# Autodesk Inventor assembly: ASSY,INTAKE
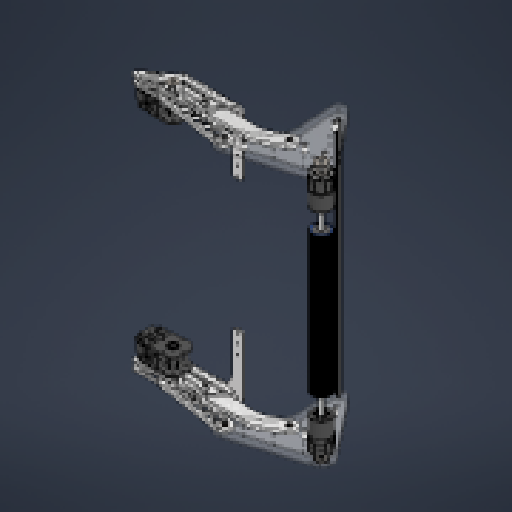
[picture p0: Inventor's stored thumbnail of the model, 512x512]
Saved by Autodesk Inventor 2026.1 (Build 301233020, 233B)
## iProperties
Created: 2026-02-09
Part Number: ASSY,INTAKE
Document SubType Name: Assembly
Designer: Jthib
Mass: 4084.96 g
Surface Area: 8083.76 cm^2
Volume: 1639.15 cm^3
Density: 2.49213 g/cm^3
Author: Jthib
## Documents named in this file (19)
- C:\Users\Owen\Documents\GitHub\2026-Robot-Mechanical\Intake\ASSY,INTAKE.iam
- C:\Users\Owen\Documents\GitHub\2026-Robot-Mechanical\Intake\PLATE,INTAKE,SIDE.ipt
- C:\Users\Owen\Documents\GitHub\2026-Robot-Mechanical\#1_CAD Library\Power Transmission\Bearings\PURCHASED,HEX_BEARING.ipt
- C:\Users\Owen\Documents\GitHub\2026-Robot-Mechanical\Intake\3DPRINT,INTAKE,SPACER.ipt
- C:\Users\Owen\Documents\GitHub\2026-Robot-Mechanical\Intake\STOCK,HEX,INTAKE.ipt
- C:\Users\Owen\Documents\GitHub\2026-Robot-Mechanical\Intake\PURCHASED,92320A546_18-8 Stainless Steel Unthreaded Spacer.ipt
- C:\Users\Owen\Documents\GitHub\2026-Robot-Mechanical\#1_CAD Library\Electronics\CONTROLS,SPARK_FLEX.ipt
- C:\Users\Owen\Documents\GitHub\2026-Robot-Mechanical\#1_CAD Library\Motors\MOTOR,REV,NEO,VORTEX.ipt
- C:\Users\Owen\Documents\GitHub\2026-Robot-Mechanical\Intake\STOCK,CHURRO,LOWER,INTAKE.ipt
- C:\Users\Owen\Documents\GitHub\2026-Robot-Mechanical\Intake\PLATE,HINGE,INTAKE,FRONT.ipt
- C:\Users\Owen\Documents\GitHub\2026-Robot-Mechanical\Intake\PLATE,LINK,FRONT,INTAKE.ipt
- C:\Users\Owen\Documents\GitHub\2026-Robot-Mechanical\Intake\PLATE,LINK,REAR,INTAKE.ipt
- C:\Users\Owen\Documents\GitHub\2026-Robot-Mechanical\Intake\PURCHASED,20-1,90deg,MAX-PLANETARY.ipt
- C:\Users\Owen\Documents\GitHub\2026-Robot-Mechanical\Intake\PURCHASED,6391K186_Oil-Embedded 841 Bronze Sleeve Bearing.ipt
- C:\Users\Owen\Documents\GitHub\2026-Robot-Mechanical\Intake\PURCHASED,92390A271_18-8 Stainless Steel Clevis Pin.ipt
- C:\Users\Owen\Documents\GitHub\2026-Robot-Mechanical\Intake\3DPRINT,SPACER,HEX,INTAKE.ipt
- C:\Users\Owen\Documents\GitHub\2026-Robot-Mechanical\Intake\PURCHASED,2796T12_Ultra-Low-Friction Dry-Running Thrust Bearing.ipt
- C:\Users\Owen\Documents\GitHub\2026-Robot-Mechanical\Intake\PLATE,CLAMP,MK4i,Swerve,CUSTOM,FRC2026.ipt
- C:\Users\Owen\Documents\GitHub\2026-Robot-Mechanical\Intake\CAST,2inOD,ROLLER.ipt
## Components (56 placed, 18 different names)
1. PLATE,INTAKE,SIDE:1 — Symmetry:1, Insert:28, Insert:29, Insert:30, Mate:31
2. PLATE,INTAKE,SIDE:2 — Angle:3, Insert:27, Mate:30
3. 3DPRINT,INTAKE,SPACER:2 — Mate:31
4. 3DPRINT,INTAKE,SPACER:4
5. 3DPRINT,INTAKE,SPACER:5
6. 3DPRINT,INTAKE,SPACER:1
7. PLATE,INTAKE,SIDE:3 — Angle:2, Insert:26, Mate:27, Mate:28, Mate:29
8. PLATE,INTAKE,SIDE:4 — Symmetry:1, Mate:8, Mate:9, Mate:10, Insert:25, Mate:33, Mate:35, Mate:50
9. 3DPRINT,INTAKE,SPACER:7 — Mate:27, Mate:28
10. 3DPRINT,INTAKE,SPACER:10
11. 3DPRINT,INTAKE,SPACER:11
12. STOCK,HEX,INTAKE:1 — Flush:1, Mate:21, Mate:22, Mate:26, Mate:63, Mate:64, Mate:65
13. PURCHASED,92320A546_18-8 Stainless Steel Unthreaded Spacer:1 — Mate:8, Mate:43
14. PURCHASED,92320A546_18-8 Stainless Steel Unthreaded Spacer:2 — Mate:9, Mate:10, Mate:23, Mate:29, Mate:46
15. MOTOR,REV,NEO,VORTEX:1 — Angle:2
16. CONTROLS,SPARK_FLEX:1
17. MOTOR,REV,NEO,VORTEX:2
18. CONTROLS,SPARK_FLEX:2 — Angle:3, Mate:26
19. PURCHASED,HEX_BEARING:7 — Insert:25, Mate:21
20. PURCHASED,HEX_BEARING:8 — Insert:26
21. PURCHASED,HEX_BEARING:9 — Insert:27
22. PURCHASED,HEX_BEARING:10 — Insert:28, Mate:22
23. PURCHASED,92320A546_18-8 Stainless Steel Unthreaded Spacer:3 — Insert:30, Mate:61
24. PURCHASED,92320A546_18-8 Stainless Steel Unthreaded Spacer:4 — Insert:29, Mate:23, Mate:30, Mate:60
25. STOCK,CHURRO,LOWER,INTAKE:1
26. PLATE,HINGE,INTAKE,FRONT:1 — Mate:38, Mate:39, Mate:48, Mate:49, Insert:40, Mate:69, Mate:70, Mate:73
27. PLATE,LINK,FRONT,INTAKE:1 — Insert:33, Insert:36
28. PLATE,LINK,REAR,INTAKE:1 — Insert:34, Mate:41
29. PURCHASED,20-1,90deg,MAX-PLANETARY:1 — Mate:69, Mate:70, Mate:73
30. PURCHASED,6391K186_Oil-Embedded 841 Bronze Sleeve Bearing:1 — Insert:33, Mate:33, Mate:43
31. PURCHASED,92390A271_18-8 Stainless Steel Clevis Pin:1 — Insert:49, Mate:66
32. PLATE,HINGE,INTAKE,FRONT:2 — Mate:38, Mate:40, Insert:39, Mate:41, Mate:42, Mate:45, Mate:47, Insert:49
33. PURCHASED,6391K186_Oil-Embedded 841 Bronze Sleeve Bearing:2 — Insert:34, Mate:35, Mate:46
34. PURCHASED,HEX_BEARING:11 — Insert:39
35. PURCHASED,6391K186_Oil-Embedded 841 Bronze Sleeve Bearing:3 — Insert:36, Insert:37, Insert:38, Mate:66
36. 3DPRINT,SPACER,HEX,INTAKE:1 — Insert:40
37. PURCHASED,2796T12_Ultra-Low-Friction Dry-Running Thrust Bearing:1 — Insert:38, Mate:39
38. PURCHASED,2796T12_Ultra-Low-Friction Dry-Running Thrust Bearing:2 — Insert:37, Mate:40
39. PLATE,CLAMP,MK4i,Swerve,CUSTOM,FRC2026:1 — Mate:47, Mate:48, Mate:49, Mate:50, Flush:5, Mate:62
40. PLATE,CLAMP,MK4i,Swerve,CUSTOM,FRC2026:2 — Flush:5, Mate:57, Mate:58, Flush:7, Mate:62
41. PLATE,HINGE,INTAKE,FRONT:3 — Mate:51, Mate:52, Insert:41, Mate:57, Mate:58, Mate:71, Insert:51, Mate:72, Mate:74
42. PLATE,HINGE,INTAKE,FRONT:4 — Mate:51, Mate:52, Insert:42, Insert:43, Mate:56, Flush:7, Insert:50
43. PLATE,LINK,REAR,INTAKE:2 — Insert:46, Mate:56, Flush:4
44. PLATE,LINK,FRONT,INTAKE:2 — Insert:44, Insert:45, Flush:4
45. PURCHASED,6391K186_Oil-Embedded 841 Bronze Sleeve Bearing:4 — Insert:44, Mate:53, Mate:54, Mate:55
46. PURCHASED,6391K186_Oil-Embedded 841 Bronze Sleeve Bearing:5 — Insert:45, Mate:61
47. PURCHASED,6391K186_Oil-Embedded 841 Bronze Sleeve Bearing:6 — Insert:46, Mate:60
48. PURCHASED,2796T12_Ultra-Low-Friction Dry-Running Thrust Bearing:3 — Insert:41, Mate:54
49. PURCHASED,2796T12_Ultra-Low-Friction Dry-Running Thrust Bearing:4 — Insert:42, Mate:55
50. PURCHASED,92390A271_18-8 Stainless Steel Clevis Pin:2 — Insert:43, Mate:53
51. CAST,2inOD,ROLLER:1 — Mate:63, Mate:68
52. CAST,2inOD,ROLLER:2 — Mate:64, Mate:67, Mate:68
53. CAST,2inOD,ROLLER:3 — Mate:65, Mate:67
54. PURCHASED,20-1,90deg,MAX-PLANETARY:2 — Mate:71, Mate:72, Mate:74
55. PURCHASED,HEX_BEARING:12 — Insert:50
56. 3DPRINT,SPACER,HEX,INTAKE:2 — Insert:51
## Relationships (97: Mate 59, Insert 31, Flush 4, Angle 2, Symmetry 1)
- [Insert]: PLATE,INTAKE,SIDE:2 ↔ 3DPRINT,INTAKE,SPACER:1
- [Insert]: PLATE,INTAKE,SIDE:2 ↔ 3DPRINT,INTAKE,SPACER:2
- [Insert]: PLATE,INTAKE,SIDE:2 ↔ 3DPRINT,INTAKE,SPACER:4
- [Insert]: PLATE,INTAKE,SIDE:2 ↔ 3DPRINT,INTAKE,SPACER:5
- [Insert]: PLATE,INTAKE,SIDE:4 ↔ 3DPRINT,INTAKE,SPACER:7
- [Insert]: PLATE,INTAKE,SIDE:4 ↔ 3DPRINT,INTAKE,SPACER:10
- [Insert]: PLATE,INTAKE,SIDE:4 ↔ 3DPRINT,INTAKE,SPACER:11
- Symmetry:1: PLATE,INTAKE,SIDE:1 ↔ PLATE,INTAKE,SIDE:4
- Flush:1: STOCK,HEX,INTAKE:1
- [Mate]: PLATE,INTAKE,SIDE:3 ↔ PURCHASED,92320A546_18-8 Stainless Steel Unthreaded Spacer:1
- Mate:8: PLATE,INTAKE,SIDE:4 ↔ PURCHASED,92320A546_18-8 Stainless Steel Unthreaded Spacer:1
- Mate:9: PLATE,INTAKE,SIDE:4 ↔ PURCHASED,92320A546_18-8 Stainless Steel Unthreaded Spacer:2
- Mate:10: PLATE,INTAKE,SIDE:4 ↔ PURCHASED,92320A546_18-8 Stainless Steel Unthreaded Spacer:2
- [Mate]: MOTOR,REV,NEO,VORTEX:1 ↔ CONTROLS,SPARK_FLEX:1
- [Mate]: MOTOR,REV,NEO,VORTEX:1 ↔ CONTROLS,SPARK_FLEX:1
- [Mate]: MOTOR,REV,NEO,VORTEX:1 ↔ CONTROLS,SPARK_FLEX:1
- [Mate]: STOCK,HEX,INTAKE:1 ↔ CONTROLS,SPARK_FLEX:1
- [Mate]: PLATE,INTAKE,SIDE:3 ↔ CONTROLS,SPARK_FLEX:1
- [Mate]: MOTOR,REV,NEO,VORTEX:2 ↔ CONTROLS,SPARK_FLEX:2
- [Mate]: MOTOR,REV,NEO,VORTEX:2 ↔ CONTROLS,SPARK_FLEX:2
- [Mate]: MOTOR,REV,NEO,VORTEX:2 ↔ CONTROLS,SPARK_FLEX:2
- [Mate]: PLATE,INTAKE,SIDE:2 ↔ CONTROLS,SPARK_FLEX:2
- Angle:2 (0 deg): PLATE,INTAKE,SIDE:3 ↔ MOTOR,REV,NEO,VORTEX:1
- Angle:3 (0 deg): PLATE,INTAKE,SIDE:2 ↔ CONTROLS,SPARK_FLEX:2
- Insert:25: PLATE,INTAKE,SIDE:4 ↔ PURCHASED,HEX_BEARING:7
- Insert:26: PLATE,INTAKE,SIDE:3 ↔ PURCHASED,HEX_BEARING:8
- Insert:27: PLATE,INTAKE,SIDE:2 ↔ PURCHASED,HEX_BEARING:9
- Insert:28: PLATE,INTAKE,SIDE:1 ↔ PURCHASED,HEX_BEARING:10
- Mate:21: STOCK,HEX,INTAKE:1 ↔ PURCHASED,HEX_BEARING:7
- Mate:22: STOCK,HEX,INTAKE:1 ↔ PURCHASED,HEX_BEARING:10
- Insert:29: PLATE,INTAKE,SIDE:1 ↔ PURCHASED,92320A546_18-8 Stainless Steel Unthreaded Spacer:4
- Insert:30: PLATE,INTAKE,SIDE:1 ↔ PURCHASED,92320A546_18-8 Stainless Steel Unthreaded Spacer:3
- Mate:23: PURCHASED,92320A546_18-8 Stainless Steel Unthreaded Spacer:2 ↔ PURCHASED,92320A546_18-8 Stainless Steel Unthreaded Spacer:4
- Mate:26: STOCK,HEX,INTAKE:1 ↔ CONTROLS,SPARK_FLEX:2
- Mate:27: PLATE,INTAKE,SIDE:3 ↔ 3DPRINT,INTAKE,SPACER:7
- Mate:28: PLATE,INTAKE,SIDE:3 ↔ 3DPRINT,INTAKE,SPACER:7
- Mate:29: PLATE,INTAKE,SIDE:3 ↔ PURCHASED,92320A546_18-8 Stainless Steel Unthreaded Spacer:2
- Mate:30: PLATE,INTAKE,SIDE:2 ↔ PURCHASED,92320A546_18-8 Stainless Steel Unthreaded Spacer:4
- Mate:31: PLATE,INTAKE,SIDE:1 ↔ 3DPRINT,INTAKE,SPACER:2
- [Insert]: PLATE,INTAKE,SIDE:3 ↔ STOCK,CHURRO,LOWER,INTAKE:1
- [Insert]: PLATE,INTAKE,SIDE:2 ↔ STOCK,CHURRO,LOWER,INTAKE:1
- Insert:33: PLATE,LINK,FRONT,INTAKE:1 ↔ PURCHASED,6391K186_Oil-Embedded 841 Bronze Sleeve Bearing:1
- Mate:33 (3.175 mm): PLATE,INTAKE,SIDE:4 ↔ PURCHASED,6391K186_Oil-Embedded 841 Bronze Sleeve Bearing:1
- Insert:34: PLATE,LINK,REAR,INTAKE:1 ↔ PURCHASED,6391K186_Oil-Embedded 841 Bronze Sleeve Bearing:2
- Mate:35 (3.175 mm): PLATE,INTAKE,SIDE:4 ↔ PURCHASED,6391K186_Oil-Embedded 841 Bronze Sleeve Bearing:2
- Insert:36: PLATE,LINK,FRONT,INTAKE:1 ↔ PURCHASED,6391K186_Oil-Embedded 841 Bronze Sleeve Bearing:3
- Insert:37: PURCHASED,6391K186_Oil-Embedded 841 Bronze Sleeve Bearing:3 ↔ PURCHASED,2796T12_Ultra-Low-Friction Dry-Running Thrust Bearing:2
- Insert:38: PURCHASED,6391K186_Oil-Embedded 841 Bronze Sleeve Bearing:3 ↔ PURCHASED,2796T12_Ultra-Low-Friction Dry-Running Thrust Bearing:1
- Mate:38: PLATE,HINGE,INTAKE,FRONT:1 ↔ PLATE,HINGE,INTAKE,FRONT:2
- Mate:39: PLATE,HINGE,INTAKE,FRONT:1 ↔ PURCHASED,2796T12_Ultra-Low-Friction Dry-Running Thrust Bearing:1
- Mate:40: PLATE,HINGE,INTAKE,FRONT:2 ↔ PURCHASED,2796T12_Ultra-Low-Friction Dry-Running Thrust Bearing:2
- Insert:39: PLATE,HINGE,INTAKE,FRONT:2 ↔ PURCHASED,HEX_BEARING:11
- Mate:41: PLATE,LINK,REAR,INTAKE:1 ↔ PLATE,HINGE,INTAKE,FRONT:2
- Mate:42: PLATE,HINGE,INTAKE,FRONT:2
- Mate:43: PURCHASED,92320A546_18-8 Stainless Steel Unthreaded Spacer:1 ↔ PURCHASED,6391K186_Oil-Embedded 841 Bronze Sleeve Bearing:1
- Mate:45: PLATE,HINGE,INTAKE,FRONT:2
- Mate:46: PURCHASED,92320A546_18-8 Stainless Steel Unthreaded Spacer:2 ↔ PURCHASED,6391K186_Oil-Embedded 841 Bronze Sleeve Bearing:2
- Mate:47: PLATE,HINGE,INTAKE,FRONT:2 ↔ PLATE,CLAMP,MK4i,Swerve,CUSTOM,FRC2026:1
- Mate:48: PLATE,HINGE,INTAKE,FRONT:1 ↔ PLATE,CLAMP,MK4i,Swerve,CUSTOM,FRC2026:1
- Mate:49 (0.1905 mm): PLATE,HINGE,INTAKE,FRONT:1 ↔ PLATE,CLAMP,MK4i,Swerve,CUSTOM,FRC2026:1
- Mate:50 (-130.175 mm): PLATE,INTAKE,SIDE:4 ↔ PLATE,CLAMP,MK4i,Swerve,CUSTOM,FRC2026:1
- Insert:40: PLATE,HINGE,INTAKE,FRONT:1 ↔ 3DPRINT,SPACER,HEX,INTAKE:1
- Mate:51: PLATE,HINGE,INTAKE,FRONT:3 ↔ PLATE,HINGE,INTAKE,FRONT:4
- Mate:52: PLATE,HINGE,INTAKE,FRONT:3 ↔ PLATE,HINGE,INTAKE,FRONT:4
- Insert:41: PLATE,HINGE,INTAKE,FRONT:3 ↔ PURCHASED,2796T12_Ultra-Low-Friction Dry-Running Thrust Bearing:3
- Insert:42: PLATE,HINGE,INTAKE,FRONT:4 ↔ PURCHASED,2796T12_Ultra-Low-Friction Dry-Running Thrust Bearing:4
- Insert:43: PLATE,HINGE,INTAKE,FRONT:4 ↔ PURCHASED,92390A271_18-8 Stainless Steel Clevis Pin:2
- Insert:44: PLATE,LINK,FRONT,INTAKE:2 ↔ PURCHASED,6391K186_Oil-Embedded 841 Bronze Sleeve Bearing:4
- Insert:45: PLATE,LINK,FRONT,INTAKE:2 ↔ PURCHASED,6391K186_Oil-Embedded 841 Bronze Sleeve Bearing:5
- Insert:46: PLATE,LINK,REAR,INTAKE:2 ↔ PURCHASED,6391K186_Oil-Embedded 841 Bronze Sleeve Bearing:6
- Mate:53: PURCHASED,6391K186_Oil-Embedded 841 Bronze Sleeve Bearing:4 ↔ PURCHASED,92390A271_18-8 Stainless Steel Clevis Pin:2
- Mate:54: PURCHASED,6391K186_Oil-Embedded 841 Bronze Sleeve Bearing:4 ↔ PURCHASED,2796T12_Ultra-Low-Friction Dry-Running Thrust Bearing:3
- Mate:55: PURCHASED,6391K186_Oil-Embedded 841 Bronze Sleeve Bearing:4 ↔ PURCHASED,2796T12_Ultra-Low-Friction Dry-Running Thrust Bearing:4
- Mate:56: PLATE,HINGE,INTAKE,FRONT:4 ↔ PLATE,LINK,REAR,INTAKE:2
- Flush:4: PLATE,LINK,REAR,INTAKE:2 ↔ PLATE,LINK,FRONT,INTAKE:2
- Flush:5: PLATE,CLAMP,MK4i,Swerve,CUSTOM,FRC2026:1 ↔ PLATE,CLAMP,MK4i,Swerve,CUSTOM,FRC2026:2
- Mate:57: PLATE,CLAMP,MK4i,Swerve,CUSTOM,FRC2026:2 ↔ PLATE,HINGE,INTAKE,FRONT:3
- Mate:58 (0.1905 mm): PLATE,CLAMP,MK4i,Swerve,CUSTOM,FRC2026:2 ↔ PLATE,HINGE,INTAKE,FRONT:3
- Flush:7: PLATE,CLAMP,MK4i,Swerve,CUSTOM,FRC2026:2 ↔ PLATE,HINGE,INTAKE,FRONT:4
- Mate:60: PURCHASED,92320A546_18-8 Stainless Steel Unthreaded Spacer:4 ↔ PURCHASED,6391K186_Oil-Embedded 841 Bronze Sleeve Bearing:6
- Mate:61: PURCHASED,92320A546_18-8 Stainless Steel Unthreaded Spacer:3 ↔ PURCHASED,6391K186_Oil-Embedded 841 Bronze Sleeve Bearing:5
- Mate:62 (-698.5 mm): PLATE,CLAMP,MK4i,Swerve,CUSTOM,FRC2026:1 ↔ PLATE,CLAMP,MK4i,Swerve,CUSTOM,FRC2026:2
- Mate:63: STOCK,HEX,INTAKE:1 ↔ CAST,2inOD,ROLLER:1
- Mate:64: STOCK,HEX,INTAKE:1 ↔ CAST,2inOD,ROLLER:2
- Mate:65: STOCK,HEX,INTAKE:1 ↔ CAST,2inOD,ROLLER:3
- Insert:49: PURCHASED,92390A271_18-8 Stainless Steel Clevis Pin:1 ↔ PLATE,HINGE,INTAKE,FRONT:2
- Mate:66: PURCHASED,92390A271_18-8 Stainless Steel Clevis Pin:1 ↔ PURCHASED,6391K186_Oil-Embedded 841 Bronze Sleeve Bearing:3
- Mate:67: CAST,2inOD,ROLLER:2 ↔ CAST,2inOD,ROLLER:3
- Mate:68: CAST,2inOD,ROLLER:1 ↔ CAST,2inOD,ROLLER:2
- Mate:69: PLATE,HINGE,INTAKE,FRONT:1 ↔ PURCHASED,20-1,90deg,MAX-PLANETARY:1
- Mate:70: PLATE,HINGE,INTAKE,FRONT:1 ↔ PURCHASED,20-1,90deg,MAX-PLANETARY:1
- Mate:71: PLATE,HINGE,INTAKE,FRONT:3 ↔ PURCHASED,20-1,90deg,MAX-PLANETARY:2
- Insert:50: PLATE,HINGE,INTAKE,FRONT:4 ↔ PURCHASED,HEX_BEARING:12
- Insert:51: PLATE,HINGE,INTAKE,FRONT:3 ↔ 3DPRINT,SPACER,HEX,INTAKE:2
- Mate:72: PLATE,HINGE,INTAKE,FRONT:3 ↔ PURCHASED,20-1,90deg,MAX-PLANETARY:2
- Mate:73: PLATE,HINGE,INTAKE,FRONT:1 ↔ PURCHASED,20-1,90deg,MAX-PLANETARY:1
- Mate:74: PLATE,HINGE,INTAKE,FRONT:3 ↔ PURCHASED,20-1,90deg,MAX-PLANETARY:2
## Named parameters: d12_d66 = 0 mm, d16_d65 = 0 mm, d19_d60 = 0 mm, d41_d26 = 0 mm, d91_d27 = 0 mm, d94_d25 = 0 mm, d95_d26 = 0 mm, d96_d91_d27 = 0 mm
